# Autodesk Inventor assembly: tip_3_ass
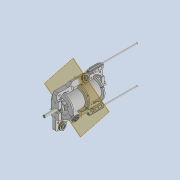
[picture p0: Inventor's stored thumbnail of the model, 180x180]
Saved by Autodesk Inventor 2020 (Build 240168000, 168)
## iProperties
Created: 2021-09-09
Part Number: tip_3_ass
Document SubType Name: Assembly
Designer: Shuang Peng
Author: Shuang Peng
## Documents named in this file (8)
- D:\projects-3\torque fb tip\hardware\tip_3\tip_3_ass.iam
- D:\projects-3\torque fb tip\hardware\tip_3\roller_1.ipt
- D:\projects-3\torque fb tip\hardware\tip_3\pin_3_30.ipt
- D:\projects-3\torque fb tip\hardware\tip_3\bearing_3_6_2.ipt
- D:\projects-3\torque fb tip\hardware\tip_3\bearing_hh_1.ipt
- D:\projects-3\torque fb tip\hardware\tip_3\ext_shell_1.ipt
- D:\projects-3\torque fb tip\hardware\tip_3\c_roller_1.ipt
- D:\projects-3\torque fb tip\hardware\tip_3\bw_ass_1.iam
## Components (17 placed, 7 different names)
1. roller_1:1 — Insert:1, Insert:2, Insert:4
2. roller_1:2 — Insert:1, Insert:3, Insert:5, Flush:5
3. pin_3_30:1 — Insert:3
4. pin_3_30:2 — Insert:2
5. bearing_3_6_2:1 — Insert:4, Flush:1
6. bearing_hh_1:1 — Flush:1, Flush:3, Flush:4
7. bearing_3_6_2:2 — Insert:5, Insert:6
8. bearing_hh_1:2 — Insert:6, Flush:3, Insert:7
9. ext_shell_1:1 — Flush:4, Insert:7, Angle:1, Insert:8, Insert:9, Insert:13, Mate:1, Flush:8, Insert:14, Mate:2, Flush:9, Mate:3
10. bearing_3_6_2:3 — Insert:9, Insert:11
11. bearing_3_6_2:4 — Insert:8, Flush:7, Insert:10
12. c_roller_1:1 — Flush:7, Insert:10
13. c_roller_1:2 — Insert:11
14. bearing_3_6_2:5 — Insert:13
15. c_roller_1:3
16. bw_ass_1:1 [sub-assembly] — Mate:1, Flush:8, Insert:14
17. bw_ass_1:2 [sub-assembly] — Mate:2, Flush:9, Mate:3
## Relationships (26: Insert 14, Flush 8, Mate 3, Angle 1)
- Insert:1: roller_1:1 ↔ roller_1:2
- Insert:2 (-20 mm): roller_1:1 ↔ pin_3_30:2
- Insert:3 (-10 mm): roller_1:2 ↔ pin_3_30:1
- Insert:4: roller_1:1 ↔ bearing_3_6_2:1
- Flush:1: bearing_3_6_2:1 ↔ bearing_hh_1:1
- [Flush]: bearing_3_6_2:2 ↔ bearing_hh_1:2
- Insert:5: roller_1:2 ↔ bearing_3_6_2:2
- Insert:6: bearing_3_6_2:2 ↔ bearing_hh_1:2
- Flush:3: bearing_hh_1:1 ↔ bearing_hh_1:2
- Flush:4: bearing_hh_1:1 ↔ ext_shell_1:1
- Insert:7: bearing_hh_1:2 ↔ ext_shell_1:1
- Angle:1 (0 deg): ext_shell_1:1
- Flush:5: roller_1:2
- Insert:8: ext_shell_1:1 ↔ bearing_3_6_2:4
- Insert:9: ext_shell_1:1 ↔ bearing_3_6_2:3
- Flush:7: bearing_3_6_2:4 ↔ c_roller_1:1
- Insert:10: bearing_3_6_2:4 ↔ c_roller_1:1
- Insert:11: bearing_3_6_2:3 ↔ c_roller_1:2
- [Insert]: bearing_3_6_2:5 ↔ c_roller_1:3
- Insert:13: ext_shell_1:1 ↔ bearing_3_6_2:5
- Mate:1: ext_shell_1:1 ↔ bw_ass_1:1
- Flush:8: ext_shell_1:1 ↔ bw_ass_1:1
- Insert:14: ext_shell_1:1 ↔ bw_ass_1:1
- Mate:2: ext_shell_1:1 ↔ bw_ass_1:2
- Flush:9: ext_shell_1:1 ↔ bw_ass_1:2
- Mate:3 (1.5 mm): ext_shell_1:1 ↔ bw_ass_1:2
## Named parameters: d5_d4 = 0 mm, d19_d18 = 0 mm
